# Autodesk Inventor assembly: Ensemble Tige-Tunel
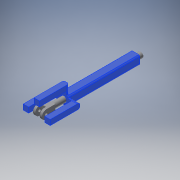
[picture p0: Inventor's stored thumbnail of the model, 180x180]
Saved by Autodesk Inventor 2018 (Build 220112000, 112)
## iProperties
Created: 2018-03-31
Part Number: Ensemble Tige-Tunel
Material: Générique
Document SubType Name: Assembly
Designer: Guadalix
Author: Guadalix
## Documents named in this file (3)
- C:\Users\Guadalix\Documents\CiP2\Semestre 2\Arduino\BARDUINO\Piezas pa imprimir en 3D\Ensemble Tige-Tunel.iam
- C:\Users\Guadalix\Documents\CiP2\Semestre 2\Arduino\BARDUINO\Piezas pa imprimir en 3D\Tunel.ipt
- C:\Users\Guadalix\Documents\CiP2\Semestre 2\Arduino\BARDUINO\Piezas pa imprimir en 3D\Tige.ipt
## Components (2 placed, 2 different names)
1. Tunel:1 — Placage:1, Affleurement:1
2. Tige:1 — Placage:1, Affleurement:1
## Relationships (2: Mate 1, Flush 1)
- Placage:1 [Mate]: Tunel:1 ↔ Tige:1
- Affleurement:1 [Flush]: Tunel:1 ↔ Tige:1
